# Autodesk Inventor assembly: mould_base_v3_p1
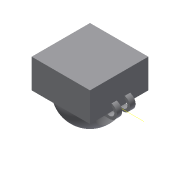
[picture p0: Inventor's stored thumbnail of the model, 180x180]
Saved by Autodesk Inventor 2017 (Build 210142000, 142)
## iProperties
Created: 2018-07-07
Part Number: mould_base_v3_p1
Document SubType Name: Assembly
Designer: Nic
Author: Nic
## Documents named in this file (4)
- C:\Users\Nic\Documents\Antenna\mould_base_v3_p1.iam
- C:\Users\Nic\Documents\Antenna\mould_casing.ipt
- C:\Users\Nic\Documents\Antenna\middle_segment_v3.ipt
- C:\Users\Nic\Documents\Antenna\sensor_pad_small.ipt
## Components (3 placed, 3 different names)
1. mould_casing:1 — Ball:1, Angle:1, Angle:2
2. middle_segment_v3:1 — Mate:1, Flush:1, Angle:2
3. sensor_pad_small:1 — Ball:1, Angle:1, Mate:1, Flush:1
## Relationships (5: Angle 2, BallJoint 1, Mate 1, Flush 1)
- Ball:1: mould_casing:1 ↔ sensor_pad_small:1
- Angle:1 (0 deg): mould_casing:1 ↔ sensor_pad_small:1
- Mate:1: middle_segment_v3:1 ↔ sensor_pad_small:1
- Flush:1 (1 mm): middle_segment_v3:1 ↔ sensor_pad_small:1
- Angle:2 (0 deg): mould_casing:1 ↔ middle_segment_v3:1
